# Autodesk Inventor assembly: flapper for sorter
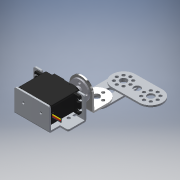
[picture p0: Inventor's stored thumbnail of the model, 180x180]
Saved by Autodesk Inventor 2019 (Build 230136000, 136)
## iProperties
Created: 2018-11-20
Part Number: flapper for sorter
Document SubType Name: Assembly
Designer: User
Author: User
## Documents named in this file (5)
- C:\Robotics\CAD\2018-19_CAD\Collection\flapper for sorter.iam
- C:\Robotics\CAD\COTSParts\Tetrix\39197_txm-485hb standard servo with horn.ipt
- C:\Robotics\CAD\COTSParts\Tetrix\39060_txm-standard servo bracket.ipt
- C:\Robotics\CAD\COTSParts\Tetrix\Tetrix bracket - angle.ipt
- C:\Robotics\CAD\COTSParts\Tetrix\39274_txm-flat64mmx27mm.ipt
## Components (5 placed, 4 different names)
1. 39197_txm-485hb standard servo with horn:1 — Mate:1, Mate:2, Mate:3, Mate:4, Mate:5
2. 39060_txm-standard servo bracket:1 — Mate:1, Mate:2, Mate:3
3. Tetrix bracket - angle:1 — Mate:4, Mate:5, Mate:6, Mate:7, Mate:11
4. 39274_txm-flat64mmx27mm:1 — Mate:6, Mate:7, Mate:8, Mate:9, Mate:10, Mate:11
5. 39274_txm-flat64mmx27mm:2 — Mate:8, Mate:9, Mate:10
## Relationships (11: Mate 11)
- Mate:1: 39197_txm-485hb standard servo with horn:1 ↔ 39060_txm-standard servo bracket:1
- Mate:2: 39197_txm-485hb standard servo with horn:1 ↔ 39060_txm-standard servo bracket:1
- Mate:3: 39197_txm-485hb standard servo with horn:1 ↔ 39060_txm-standard servo bracket:1
- Mate:4: 39197_txm-485hb standard servo with horn:1 ↔ Tetrix bracket - angle:1
- Mate:5: 39197_txm-485hb standard servo with horn:1 ↔ Tetrix bracket - angle:1
- Mate:6: Tetrix bracket - angle:1 ↔ 39274_txm-flat64mmx27mm:1
- Mate:7: Tetrix bracket - angle:1 ↔ 39274_txm-flat64mmx27mm:1
- Mate:8: 39274_txm-flat64mmx27mm:1 ↔ 39274_txm-flat64mmx27mm:2
- Mate:9: 39274_txm-flat64mmx27mm:1 ↔ 39274_txm-flat64mmx27mm:2
- Mate:10: 39274_txm-flat64mmx27mm:1 ↔ 39274_txm-flat64mmx27mm:2
- Mate:11: Tetrix bracket - angle:1 ↔ 39274_txm-flat64mmx27mm:1
